# Autodesk Inventor assembly: Tower Assm
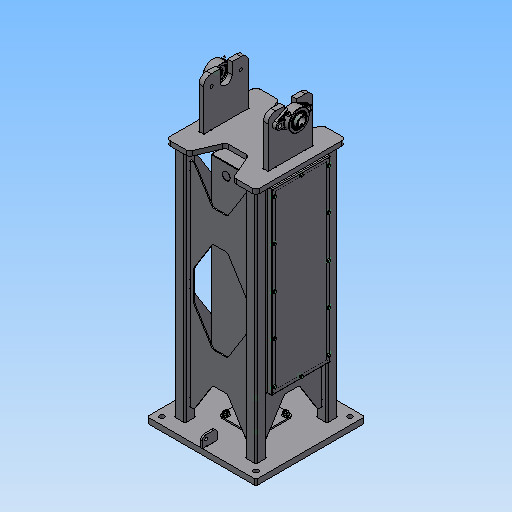
[picture p0: Inventor's stored thumbnail of the model, 512x512]
Saved by Autodesk Inventor 2025.4 (Build 294407000, 407)
## iProperties
RuleStatus: InUse
Created: 2025-09-18
Part Number: Tower Assm
Document SubType Name: Assembly
Designer: titus
Description: Cleaning Robot Tower Assembly
Mass: 62310.8 g
Surface Area: 35204 cm^2
Volume: 7937.69 cm^3
Density: 7.85 g/cm^3
Author: titus
## iProperties of the stored document MemberDocs/xCri0qr5lMkvr1sz0Uydxa0q2Qc
RuleStatus: InUse
Created: 2025-09-18
Part Number: Tower Assm
Document SubType Name: Assembly
Designer: titus
Description: Cleaning Robot Tower Assembly
Mass: 62310.8 g
Surface Area: 35204 cm^2
Volume: 7937.69 cm^3
Density: 7.85 g/cm^3
Author: titus
## Documents named in this file (17)
- R:\A1- Neuweg Design Data\OM Robotics\CLEANING ROBOT TOWER PROJECT\Tower Assm.iam
- R:\A1- Neuweg Design Data\OM Robotics\CLEANING ROBOT TOWER PROJECT\Tower Base.ipt
- R:\A1- Neuweg Design Data\OM Robotics\CLEANING ROBOT TOWER PROJECT\Tower Top Plate.ipt
- R:\A1- Neuweg Design Data\OM Robotics\CLEANING ROBOT TOWER PROJECT\Arm Mount Plate.ipt
- R:\A1- Neuweg Design Data\OM Robotics\CLEANING ROBOT TOWER PROJECT\Tower Actuator Mount Tab.ipt
- R:\A1- Neuweg Design Data\OM Robotics\CLEANING ROBOT TOWER PROJECT\Corner Post.ipt
- R:\A1- Neuweg Design Data\OM Robotics\CLEANING ROBOT TOWER PROJECT\Tower Cross Support.ipt
- R:\A1- Neuweg Design Data\OM Robotics\CLEANING ROBOT TOWER PROJECT\Corner Post 2.ipt
- R:\A1- Neuweg Design Data\OM Robotics\CLEANING ROBOT TOWER PROJECT\Corner Post 3.ipt
- R:\A1- Neuweg Design Data\OM Robotics\CLEANING ROBOT TOWER PROJECT\Corner Post 4.ipt
- R:\A1- Neuweg Design Data\OM Robotics\CLEANING ROBOT TOWER PROJECT\Half cross support.ipt
- R:\A1- Neuweg Design Data\OM Robotics\CLEANING ROBOT TOWER PROJECT\ELB-ASM-1001.iam
- R:\A1- Neuweg Design Data\OM Robotics\CLEANING ROBOT TOWER PROJECT\92979A340.ipt
- R:\A1- Neuweg Design Data\OM Robotics\CLEANING ROBOT TOWER PROJECT\ELB-ASM-1000.iam
- R:\A1- Neuweg Design Data\OM Robotics\CLEANING ROBOT TOWER PROJECT\5968K75.ipt
- R:\A1- Neuweg Design Data\OM Robotics\CLEANING ROBOT TOWER PROJECT\92979A114.ipt
- R:\A1- Neuweg Design Data\OM Robotics\CLEANING ROBOT TOWER PROJECT\1_4-20 UNC x 0.625.ipt
## Components (27 placed, 15 different names)
1. Tower Base — Insert:1, Insert:2
2. Tower Top Plate:1
3. Arm Mount Plate:1 — Insert:15, Insert:16
4. Tower Actuator Mount Tab:1
5. Corner Post:1
6. Arm Mount Plate:2 — Insert:17, Insert:18
7. Corner Post 2:1
8. Corner Post 3:1 — Mate:8
9. Corner Post 4:1 — Mate:7
10. Half cross support:1
11. ELB-ASM-1001:1 [sub-assembly] — Insert:1, Insert:2, Insert:3, Insert:4, Insert:5, Insert:6, Insert:7, Insert:8
12. 92979A340:1 — Insert:3
13. 92979A340:2 — Insert:4
14. 92979A340:3 — Insert:5
15. 92979A340:4 — Insert:6
16. ELB-ASM-1000:1 [sub-assembly] — Insert:7, Insert:8, Insert:9, Insert:10, Insert:11, Insert:12, Insert:13, Insert:14, Mate:7, Mate:8
17. 92979A114:1 — Insert:13
18. 92979A114:2 — Insert:14
19. 92979A114:3 — Insert:9
20. 92979A114:4 — Insert:10
21. 92979A114:5 — Insert:11
22. 92979A114:6 — Insert:12
23. 5968K75:1 — Insert:15, Insert:16
24. 5968K75:2 — Insert:17, Insert:18
25. Tower Cross Support:1
26. Tower Cross Support:2
27. Tower Cross Support:3
## Component patterns: (3 elements, first: Tower Cross Support:1)
## Relationships (23: Insert 18, Mate 3, Flush 2)
- [Mate]: Tower Top Plate:1 ↔ Arm Mount Plate:2
- [Flush]: Arm Mount Plate:1 ↔ Arm Mount Plate:2
- [Flush] (34.925 mm): Tower Top Plate:1 ↔ Arm Mount Plate:2
- Insert:1: Tower Base ↔ ELB-ASM-1001:1
- Insert:2: Tower Base ↔ ELB-ASM-1001:1
- Insert:3: ELB-ASM-1001:1 ↔ 92979A340:1
- Insert:4: ELB-ASM-1001:1 ↔ 92979A340:2
- Insert:5: ELB-ASM-1001:1 ↔ 92979A340:3
- Insert:6: ELB-ASM-1001:1 ↔ 92979A340:4
- Insert:7: ELB-ASM-1001:1 ↔ ELB-ASM-1000:1
- Insert:8: ELB-ASM-1001:1 ↔ ELB-ASM-1000:1
- Insert:9: ELB-ASM-1000:1 ↔ 92979A114:3
- Insert:10: ELB-ASM-1000:1 ↔ 92979A114:4
- Insert:11: ELB-ASM-1000:1 ↔ 92979A114:5
- Insert:12: ELB-ASM-1000:1 ↔ 92979A114:6
- Insert:13: ELB-ASM-1000:1 ↔ 92979A114:1
- Insert:14: ELB-ASM-1000:1 ↔ 92979A114:2
- Mate:7: Corner Post 4:1 ↔ ELB-ASM-1000:1
- Mate:8: Corner Post 3:1 ↔ ELB-ASM-1000:1
- Insert:15: Arm Mount Plate:1 ↔ 5968K75:1
- Insert:16: Arm Mount Plate:1 ↔ 5968K75:1
- Insert:17: Arm Mount Plate:2 ↔ 5968K75:2
- Insert:18: Arm Mount Plate:2 ↔ 5968K75:2
## Named parameters: d3_d2 = 0 mm
